# Autodesk Inventor assembly: DH_Assembly
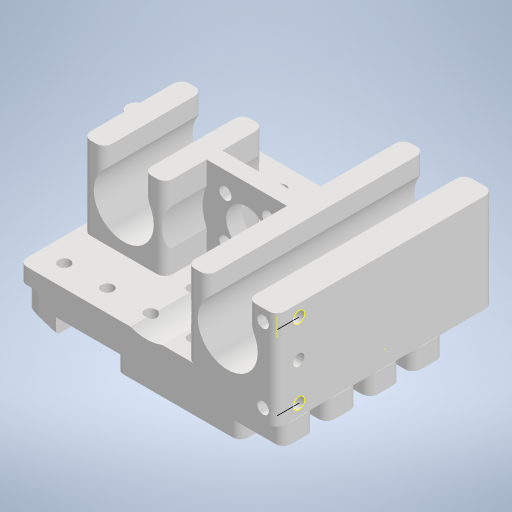
[picture p0: Inventor's stored thumbnail of the model, 512x512]
Saved by Autodesk Inventor 2023 (Build 270158000, 158)
## iProperties
Created: 2023-09-28
Part Number: DH_Assembly
Document SubType Name: Assembly
Designer: au323799
Author: au323799
## Documents named in this file (3)
- C:\Users\au323799\OneDrive - Aarhus Universitet\A_Articles\ASM_AuNP\3-Automation\Figures\CAD\DH_Assembly.iam
- C:\Users\au323799\OneDrive - Aarhus Universitet\A_Articles\ASM_AuNP\3-Automation\Figures\CAD\DH_Gantry.ipt
- C:\Users\au323799\OneDrive - Aarhus Universitet\A_Articles\ASM_AuNP\3-Automation\Figures\CAD\DH_tubing_holder.ipt
## Components (5 placed, 2 different names)
1. DH_Gantry:1 — Rotational:1, Mate:1, Mate:2, Rotational:2, Rotational:3, Rotational:4, Mate:3, Mate:4, Mate:5
2. DH_tubing_holder:1 — Rotational:1, Mate:1, Mate:2
3. DH_tubing_holder:2 — Rotational:2, Mate:3
4. DH_tubing_holder:4 — Rotational:3, Mate:5
5. DH_tubing_holder:5 — Rotational:4, Mate:4
## Relationships (9: Mate 5, RevoluteJoint 4)
- Rotational:1 [RevoluteJoint]: DH_Gantry:1 ↔ DH_tubing_holder:1
- Mate:1: DH_Gantry:1 ↔ DH_tubing_holder:1
- Mate:2: DH_Gantry:1 ↔ DH_tubing_holder:1
- Rotational:2 [RevoluteJoint]: DH_Gantry:1 ↔ DH_tubing_holder:2
- Rotational:3 [RevoluteJoint]: DH_Gantry:1 ↔ DH_tubing_holder:4
- Rotational:4 [RevoluteJoint]: DH_Gantry:1 ↔ DH_tubing_holder:5
- Mate:3: DH_Gantry:1 ↔ DH_tubing_holder:2
- Mate:4: DH_Gantry:1 ↔ DH_tubing_holder:5
- Mate:5: DH_Gantry:1 ↔ DH_tubing_holder:4
